# Autodesk Inventor assembly: vertical cyinder asm
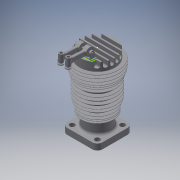
[picture p0: Inventor's stored thumbnail of the model, 180x180]
Saved by Autodesk Inventor 2018 (Build 220112000, 112)
## iProperties
Created: 2021-03-17
Part Number: vertical cyinder asm
Document SubType Name: Assembly
Designer: Jyoti Soni
Author: Jyoti Soni
## Documents named in this file (5)
- C:\Users\Jyoti Soni\Desktop\asm\15032021\vertical cyinder asm.iam
- C:\Users\Jyoti Soni\Desktop\asm\15032021\vertical cylinder.ipt
- C:\Users\Jyoti Soni\Desktop\asm\15032021\pin.ipt
- C:\Users\Jyoti Soni\Desktop\asm\15032021\knuckle.ipt
- C:\Users\Jyoti Soni\Desktop\asm\15032021\lower pin.ipt
## Components (6 placed, 4 different names)
1. vertical cylinder:1 — Mate:1, Flush:1, Mate:3, Mate:6
2. pin:1 — Mate:1, Flush:1, Mate:2, Mate:4, Mate:5
3. knuckle:1 — Mate:2, Mate:3, Mate:4, Mate:7, Mate:8
4. knuckle:2 — Mate:5, Mate:6, Mate:9, Mate:10
5. lower pin:1 — Mate:7, Mate:8
6. lower pin:2 — Mate:9, Mate:10
## Relationships (11: Mate 10, Flush 1)
- Mate:1: vertical cylinder:1 ↔ pin:1
- Flush:1 (1 mm): vertical cylinder:1 ↔ pin:1
- Mate:2: pin:1 ↔ knuckle:1
- Mate:3 (2 mm): vertical cylinder:1 ↔ knuckle:1
- Mate:4: pin:1 ↔ knuckle:1
- Mate:5: pin:1 ↔ knuckle:2
- Mate:6 (2 mm): vertical cylinder:1 ↔ knuckle:2
- Mate:7: knuckle:1 ↔ lower pin:1
- Mate:8 (2 mm): knuckle:1 ↔ lower pin:1
- Mate:9: knuckle:2 ↔ lower pin:2
- Mate:10 (2 mm): knuckle:2 ↔ lower pin:2
